# Autodesk Inventor assembly: WCP_DS_-_2_CIM_WCD_Base_Kit_217-3433
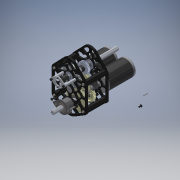
[picture p0: Inventor's stored thumbnail of the model, 180x180]
Saved by Autodesk Inventor 2017 (Build 210142000, 142)
## iProperties
Created: 2013-12-10
Part Number: WCP_DS_-_2_CIM_WCD_Base_Kit_217-3433
Description: STEP AP214
Document SubType Name: Assembly
Designer: 600086
Mass: 1467.69 g
Surface Area: 3535.67 cm^2
Volume: 1467.69 cm^3
Density: 1 g/cm^3
Sending System: SolidWorks 2013
Preprocessor: SwSTEP 2.0
Title: 217-3433-STEP.STEP
Revision Number: ANY
## Documents named in this file (43)
- E:\GrabCAD\Power Hawks CAD\Resources\VEXpro Resources\Gearboxes\WCP shifting Gearbox\WCP_DS_-_2_CIM_WCD_Base_Kit_217-3433.iam
- E:\GrabCAD\Power Hawks CAD\Resources\VEXpro Resources\Gearboxes\WCP shifting Gearbox\217-3423-005 Rev1.ipt
- E:\GrabCAD\Power Hawks CAD\Resources\VEXpro Resources\Gearboxes\WCP shifting Gearbox\217-3195-200 Rev1.iam
- E:\GrabCAD\Power Hawks CAD\Resources\VEXpro Resources\Gearboxes\WCP shifting Gearbox\217-3423-006 Rev1.ipt
- E:\GrabCAD\Power Hawks CAD\Resources\VEXpro Resources\Gearboxes\WCP shifting Gearbox\217-3423-008 Rev1.ipt
- E:\GrabCAD\Power Hawks CAD\Resources\VEXpro Resources\Gearboxes\WCP shifting Gearbox\217-3423-009 Rev1.ipt
- E:\GrabCAD\Power Hawks CAD\Resources\VEXpro Resources\Gearboxes\WCP shifting Gearbox\217-2778-001 Rev2_NCQ8A075-050M.iam
- E:\GrabCAD\Power Hawks CAD\Resources\VEXpro Resources\Gearboxes\WCP shifting Gearbox\217-2731.ipt
- E:\GrabCAD\Power Hawks CAD\Resources\VEXpro Resources\Gearboxes\WCP shifting Gearbox\217-2733.ipt
- E:\GrabCAD\Power Hawks CAD\Resources\VEXpro Resources\Gearboxes\WCP shifting Gearbox\217-2734.ipt
- E:\GrabCAD\Power Hawks CAD\Resources\VEXpro Resources\Gearboxes\WCP shifting Gearbox\217-2743.ipt
- E:\GrabCAD\Power Hawks CAD\Resources\VEXpro Resources\Gearboxes\WCP shifting Gearbox\217-2614-002_98430A132.ipt
- E:\GrabCAD\Power Hawks CAD\Resources\VEXpro Resources\Gearboxes\WCP shifting Gearbox\217-3421-007 Rev1.ipt
- E:\GrabCAD\Power Hawks CAD\Resources\VEXpro Resources\Gearboxes\WCP shifting Gearbox\217-3421-009 Rev1.ipt
- E:\GrabCAD\Power Hawks CAD\Resources\VEXpro Resources\Gearboxes\WCP shifting Gearbox\217-3421-010 Rev1.ipt
- E:\GrabCAD\Power Hawks CAD\Resources\VEXpro Resources\Gearboxes\WCP shifting Gearbox\217-3421-011 Rev2_97633A200.ipt
- E:\GrabCAD\Power Hawks CAD\Resources\VEXpro Resources\Gearboxes\WCP shifting Gearbox\217-3422-007 Rev1.ipt
- E:\GrabCAD\Power Hawks CAD\Resources\VEXpro Resources\Gearboxes\WCP shifting Gearbox\217-3423-014 Rev1.ipt
- E:\GrabCAD\Power Hawks CAD\Resources\VEXpro Resources\Gearboxes\WCP shifting Gearbox\217-3423-016 Rev1.ipt
- E:\GrabCAD\Power Hawks CAD\Resources\VEXpro Resources\Gearboxes\WCP shifting Gearbox\217-3424-003 Rev1.ipt
- E:\GrabCAD\Power Hawks CAD\Resources\VEXpro Resources\Gearboxes\WCP shifting Gearbox\217-2761-001 rev1.ipt
- E:\GrabCAD\Power Hawks CAD\Resources\VEXpro Resources\Gearboxes\WCP shifting Gearbox\217-3210-001 Rev1_30t.ipt
- E:\GrabCAD\Power Hawks CAD\Resources\VEXpro Resources\Gearboxes\WCP shifting Gearbox\217-3215-001 Rev1_42t.ipt
- E:\GrabCAD\Power Hawks CAD\Resources\VEXpro Resources\Gearboxes\WCP shifting Gearbox\217-3414-001 Rev1_14t Steel Pinion.ipt
- E:\GrabCAD\Power Hawks CAD\Resources\VEXpro Resources\Gearboxes\WCP shifting Gearbox\217-3418-001 Rev2_44t.ipt
- E:\GrabCAD\Power Hawks CAD\Resources\VEXpro Resources\Gearboxes\WCP shifting Gearbox\217-3420-001 Rev2_60t.ipt
- E:\GrabCAD\Power Hawks CAD\Resources\VEXpro Resources\Gearboxes\WCP shifting Gearbox\217-3100-001_14t.ipt
- E:\GrabCAD\Power Hawks CAD\Resources\VEXpro Resources\Gearboxes\WCP shifting Gearbox\217-2705-001_30t.ipt
- E:\GrabCAD\Power Hawks CAD\Resources\VEXpro Resources\Gearboxes\WCP shifting Gearbox\217-2000.ipt
- E:\GrabCAD\Power Hawks CAD\Resources\VEXpro Resources\Gearboxes\WCP shifting Gearbox\217-3433-001 Rev1_Default_As Machined_.ipt
- E:\GrabCAD\Power Hawks CAD\Resources\VEXpro Resources\Gearboxes\WCP shifting Gearbox\217-3423-003 Rev1.ipt
- E:\GrabCAD\Power Hawks CAD\Resources\VEXpro Resources\Gearboxes\WCP shifting Gearbox\217-3424-005 Rev1.ipt
- E:\GrabCAD\Power Hawks CAD\Resources\VEXpro Resources\Gearboxes\WCP shifting Gearbox\217-3256-001 Rev1.ipt
- E:\GrabCAD\Power Hawks CAD\Resources\VEXpro Resources\Gearboxes\WCP shifting Gearbox\217-3261-001 Rev1.ipt
- E:\GrabCAD\Power Hawks CAD\Resources\VEXpro Resources\Gearboxes\WCP shifting Gearbox\217-3423-004 Rev1.ipt
- E:\GrabCAD\Power Hawks CAD\Resources\VEXpro Resources\Gearboxes\WCP shifting Gearbox\217-3424-002 Rev1.ipt
- E:\GrabCAD\Power Hawks CAD\Resources\VEXpro Resources\Gearboxes\WCP shifting Gearbox\217-3422-004 Rev2.ipt
- E:\GrabCAD\Power Hawks CAD\Resources\VEXpro Resources\Gearboxes\WCP shifting Gearbox\217-3257-001 Rev1.ipt
- E:\GrabCAD\Power Hawks CAD\Resources\VEXpro Resources\Gearboxes\WCP shifting Gearbox\217-3263-001 Rev1.ipt
- E:\GrabCAD\Power Hawks CAD\Resources\VEXpro Resources\Gearboxes\WCP shifting Gearbox\217-3259-001 Rev1.ipt
- E:\GrabCAD\Power Hawks CAD\Resources\VEXpro Resources\Gearboxes\WCP shifting Gearbox\217-2758-001 Rev1.ipt
- E:\GrabCAD\Power Hawks CAD\Resources\VEXpro Resources\Versa Motion\Sprockets\1.125HexboreSprocket22t-ver-1111-2018.ipt
- E:\GrabCAD\Power Hawks CAD\2018 - Power Up\Chassis\pto\PTO_Add-On_Kit_217-3636.iam
## Components (71 placed, 71 different names)
1. 217-3423-005 Rev1_2 — Rigid:42, Rigid:43, Rigid:44, Rigid:45, Rotational:26
2. 217-3195-200 Rev1_3 [sub-assembly] — Rigid:46
3. 217-3423-006 Rev1_5 — Rigid:45, Rotational:49
4. 217-3423-006 Rev1_6 — Rigid:44, Rotational:48
5. 217-3423-008 Rev1_7 — Mate:4, Mate:5
6. 217-3423-009 Rev1_8 — Rotational:7, Mate:4, Mate:5, Rigid:30, Angle:2, Mate:6
7. 217-2778-001 Rev2_NCQ8A075-050M_9 [sub-assembly] — Rotational:26
8. 217-2731_10 — Rotational:24, Rigid:25, Rigid:29
9. 217-2733_11 — Rotational:4
10. 217-2733_12 — Rotational:2, Rigid:4
11. 217-2734_13 — Rotational:5, Rigid:18, Angle:4
12. 217-2734_14 — Rigid:21, Rigid:22, Cylindrical:1
13. 217-2743_15 — Rigid:24, Rigid:29, Rigid:31
14. 217-2731_16 — Rotational:1
15. 217-2731_17 — Rigid:3
16. 217-2614-002_98430A132_18 — Rigid:34
17. 217-2614-002_98430A132_19 — Rigid:35
18. 217-2614-002_98430A132_20 — Rigid:36
19. 217-2614-002_98430A132_21 — Rigid:37
20. 217-3421-007 Rev1_24 — Rigid:42
21. 217-3421-007 Rev1_25 — Rigid:43
22. 217-3421-009 Rev1_26 — Rigid:51
23. 217-3421-009 Rev1_27 — Rigid:50
24. 217-3421-009 Rev1_28 — Rigid:49
25. 217-3421-009 Rev1_29 — Rigid:52
26. 217-3421-009 Rev1_30 — Rigid:48
27. 217-3421-009 Rev1_31 — Rigid:47
28. 217-3421-010 Rev1_32 — Rigid:40
29. 217-3421-010 Rev1_33 — Rigid:39
30. 217-3421-010 Rev1_34 — Rigid:41
31. 217-3421-010 Rev1_35 — Rigid:38
32. 217-3421-011 Rev2_97633A200_36 — Rigid:26
33. 217-3422-007 Rev1_37 — Mate:7, Flush:3
34. 217-3422-007 Rev1_38 — Mate:8, Flush:2
35. 217-3423-014 Rev1_39 — Rigid:30
36. 217-3423-016 Rev1_40 — Rigid:28
37. 217-3423-016 Rev1_41 — Rigid:27
38. 217-3423-016 Rev1_42
39. 217-3424-003 Rev1_43 — Rigid:14
40. 217-3424-003 Rev1_44 — Rigid:13
41. 217-3424-003 Rev1_45 — Rigid:12
42. 217-3424-003 Rev1_46 — Rigid:11
43. 217-2761-001 rev1_47
44. 217-3210-001 Rev1_30t_50 — Rigid:9
45. 217-3215-001 Rev1_42t_51 — Rigid:8, Rigid:9, Flush:1, Rotation:1, Rotation:2, Rotation:3, Rotation:4
46. 217-3414-001 Rev1_14t Steel Pinion_52217-3414-001 Rev1_14t Steel Pinion_52 — Cylindrical:2, Rigid:34, Rigid:35, Flush:1, Rotation:1
47. 217-3418-001 Rev2_44t_55 — Rigid:24, Rotational:7, Rotation:4
48. 217-3420-001 Rev2_60t_56 — Rigid:21, Mate:6
49. 217-3100-001_14t_57 — Rigid:5, Rigid:7
50. 217-2705-001_30t_58 — Rigid:2, Rigid:53, Rotation:3
51. 217-2000_59 — Rotational:51, Cylindrical:2, Mate:10
52. 217-2000_60 — Rotational:52, Rotational:25, Mate:11
53. 217-3433-001 Rev1_Default<As Machined>_62 — Rotational:4, Rotational:24, Rigid:27, Rigid:28, Rotational:8, Rotational:9, Rotational:52, Rotational:51, Rigid:38, Rigid:39, Rigid:40, Rigid:41, Rotational:48, Rotational:49, Rigid:47, Rigid:48, Mate:10, Mate:11, Rigid:49, Rigid:50, Rigid:51, Rigid:52
54. 217-3433-001 Rev1_Default<As Machined>_63 — Rotational:1, Rotational:2, Mate:1, Mate:2, Mate:3, Rigid:11, Rigid:12, Rigid:13, Rigid:14, Rotational:6, Rigid:15, Rigid:16, Rigid:17, Rotational:56, Rotational:57
55. 217-3423-003 Rev1_64 — Rigid:31, Angle:2, Cylindrical:1, Angle:3, Angle:4, Rigid:46
56. 217-3424-005 Rev1_65 — Rigid:4, Rigid:5
57. 217-3256-001 Rev1_67 — Rigid:7, Rigid:8
58. 217-3261-001 Rev1_68 — Rigid:2, Rigid:3
59. 217-3423-004 Rev1_69 — Rigid:25, Rigid:26
60. 217-3424-002 Rev1_70 — Rigid:17
61. 217-3424-002 Rev1_71 — Rigid:16, Rotational:8
62. 217-3424-002 Rev1_72 — Rotational:6, Rotational:9
63. 217-3424-002 Rev1_73 — Rigid:15
64. 217-3422-004 Rev2_74 — Mate:1, Mate:2, Mate:3, Rotational:5, Mate:7, Mate:8, Flush:2, Flush:3
65. 217-3257-001 Rev1_75 — Rigid:22, Angle:3
66. 217-3263-001 Rev1_76 — Rigid:18, Rigid:19
67. 217-3259-001 Rev1_77 — Rigid:19, Rigid:20
68. 217-2758-001 Rev1_78 — Rigid:20
69. 217-3414-001 Rev1_14t Steel Pinion:2 — Rotational:25, Rigid:36, Rigid:37, Rotation:2
70. 1.125HexboreSprocket22t-ver-1111-2018:1 — Rotational:58, Mate:12
71. PTO_Add-On_Kit_217-3636:1 [sub-assembly] — Rotational:56, Rotational:57, Rigid:53, Rotational:58, Mate:12
## Relationships (88: WeldJoint 47, RevoluteJoint 18, Mate 11, RelateRotation 4, Angle 3, Flush 3, CylindricalJoint 2)
- Rotational:1 [RevoluteJoint]: 217-2731_16 ↔ 217-3433-001 Rev1_Default<As Machined>_63
- Rotational:2 [RevoluteJoint]: 217-2733_12 ↔ 217-3433-001 Rev1_Default<As Machined>_63
- Rigid:2 [WeldJoint]: 217-2705-001_30t_58 ↔ 217-3261-001 Rev1_68
- Rigid:3 [WeldJoint]: 217-2731_17 ↔ 217-3261-001 Rev1_68
- Rigid:4 [WeldJoint]: 217-2733_12 ↔ 217-3424-005 Rev1_65
- Rigid:5 [WeldJoint]: 217-3100-001_14t_57 ↔ 217-3424-005 Rev1_65
- Rotational:4 [RevoluteJoint]: 217-2733_11 ↔ 217-3433-001 Rev1_Default<As Machined>_62
- Rigid:7 [WeldJoint]: 217-3100-001_14t_57 ↔ 217-3256-001 Rev1_67
- Rigid:8 [WeldJoint]: 217-3215-001 Rev1_42t_51 ↔ 217-3256-001 Rev1_67
- Rigid:9 [WeldJoint]: 217-3210-001 Rev1_30t_50 ↔ 217-3215-001 Rev1_42t_51
- Mate:1: 217-3433-001 Rev1_Default<As Machined>_63 ↔ 217-3422-004 Rev2_74
- Mate:2: 217-3433-001 Rev1_Default<As Machined>_63 ↔ 217-3422-004 Rev2_74
- Mate:3: 217-3433-001 Rev1_Default<As Machined>_63 ↔ 217-3422-004 Rev2_74
- Rotational:5 [RevoluteJoint]: 217-2734_13 ↔ 217-3422-004 Rev2_74
- Rigid:11 [WeldJoint]: 217-3424-003 Rev1_46 ↔ 217-3433-001 Rev1_Default<As Machined>_63
- Rigid:12 [WeldJoint]: 217-3424-003 Rev1_45 ↔ 217-3433-001 Rev1_Default<As Machined>_63
- Rigid:13 [WeldJoint]: 217-3424-003 Rev1_44 ↔ 217-3433-001 Rev1_Default<As Machined>_63
- Rigid:14 [WeldJoint]: 217-3424-003 Rev1_43 ↔ 217-3433-001 Rev1_Default<As Machined>_63
- Rotational:6 [RevoluteJoint]: 217-3433-001 Rev1_Default<As Machined>_63 ↔ 217-3424-002 Rev1_72
- Rigid:15 [WeldJoint]: 217-3433-001 Rev1_Default<As Machined>_63 ↔ 217-3424-002 Rev1_73
- Rigid:16 [WeldJoint]: 217-3433-001 Rev1_Default<As Machined>_63 ↔ 217-3424-002 Rev1_71
- Rigid:17 [WeldJoint]: 217-3433-001 Rev1_Default<As Machined>_63 ↔ 217-3424-002 Rev1_70
- Rigid:18 [WeldJoint]: 217-2734_13 ↔ 217-3263-001 Rev1_76
- Rigid:19 [WeldJoint]: 217-3263-001 Rev1_76 ↔ 217-3259-001 Rev1_77
- Rigid:20 [WeldJoint]: 217-3259-001 Rev1_77 ↔ 217-2758-001 Rev1_78
- Rigid:21 [WeldJoint]: 217-2734_14 ↔ 217-3420-001 Rev2_60t_56
- Rigid:22 [WeldJoint]: 217-2734_14 ↔ 217-3257-001 Rev1_75
- Rotational:24 [RevoluteJoint]: 217-2731_10 ↔ 217-3433-001 Rev1_Default<As Machined>_62
- Rigid:24 [WeldJoint]: 217-2743_15 ↔ 217-3418-001 Rev2_44t_55
- Rotational:7 [RevoluteJoint]: 217-3423-009 Rev1_8 ↔ 217-3418-001 Rev2_44t_55
- Rigid:25 [WeldJoint]: 217-2731_10 ↔ 217-3423-004 Rev1_69
- Rigid:26 [WeldJoint]: 217-3421-011 Rev2_97633A200_36 ↔ 217-3423-004 Rev1_69
- Rigid:27 [WeldJoint]: 217-3423-016 Rev1_41 ↔ 217-3433-001 Rev1_Default<As Machined>_62
- Rigid:28 [WeldJoint]: 217-3423-016 Rev1_40 ↔ 217-3433-001 Rev1_Default<As Machined>_62
- Rigid:29 [WeldJoint]: 217-2731_10 ↔ 217-2743_15
- Mate:4: 217-3423-008 Rev1_7 ↔ 217-3423-009 Rev1_8
- Mate:5: 217-3423-008 Rev1_7 ↔ 217-3423-009 Rev1_8
- Rigid:30 [WeldJoint]: 217-3423-009 Rev1_8 ↔ 217-3423-014 Rev1_39
- Rigid:31 [WeldJoint]: 217-2743_15 ↔ 217-3423-003 Rev1_64
- Angle:2 (0 deg): 217-3423-009 Rev1_8 ↔ 217-3423-003 Rev1_64
- Cylindrical:1: 217-2734_14 ↔ 217-3423-003 Rev1_64
- Mate:6 (26.67 mm): 217-3423-009 Rev1_8 ↔ 217-3420-001 Rev2_60t_56
- Angle:3 (0 deg): 217-3423-003 Rev1_64 ↔ 217-3257-001 Rev1_75
- Rotational:8 [RevoluteJoint]: 217-3433-001 Rev1_Default<As Machined>_62 ↔ 217-3424-002 Rev1_71
- Rotational:9 [RevoluteJoint]: 217-3433-001 Rev1_Default<As Machined>_62 ↔ 217-3424-002 Rev1_72
- Rotational:52 [RevoluteJoint]: 217-2000_60 ↔ 217-3433-001 Rev1_Default<As Machined>_62
- Rotational:51 [RevoluteJoint]: 217-2000_59 ↔ 217-3433-001 Rev1_Default<As Machined>_62
- Cylindrical:2: 217-3414-001 Rev1_14t Steel Pinion_52217-3414-001 Rev1_14t Steel Pinion_52 ↔ 217-2000_59
- Rigid:34 [WeldJoint]: 217-2614-002_98430A132_18 ↔ 217-3414-001 Rev1_14t Steel Pinion_52217-3414-001 Rev1_14t Steel Pinion_52
- Rigid:35 [WeldJoint]: 217-2614-002_98430A132_19 ↔ 217-3414-001 Rev1_14t Steel Pinion_52217-3414-001 Rev1_14t Steel Pinion_52
- Flush:1: 217-3215-001 Rev1_42t_51 ↔ 217-3414-001 Rev1_14t Steel Pinion_52217-3414-001 Rev1_14t Steel Pinion_52
- Rotational:25 [RevoluteJoint]: 217-2000_60 ↔ 217-3414-001 Rev1_14t Steel Pinion:2
- Rigid:36 [WeldJoint]: 217-2614-002_98430A132_20 ↔ 217-3414-001 Rev1_14t Steel Pinion:2
- Rigid:37 [WeldJoint]: 217-2614-002_98430A132_21 ↔ 217-3414-001 Rev1_14t Steel Pinion:2
- Mate:7: 217-3422-007 Rev1_37 ↔ 217-3422-004 Rev2_74
- Mate:8: 217-3422-007 Rev1_38 ↔ 217-3422-004 Rev2_74
- Flush:2: 217-3422-007 Rev1_38 ↔ 217-3422-004 Rev2_74
- Flush:3: 217-3422-007 Rev1_37 ↔ 217-3422-004 Rev2_74
- Angle:4 (0 deg): 217-2734_13 ↔ 217-3423-003 Rev1_64
- Rigid:38 [WeldJoint]: 217-3421-010 Rev1_35 ↔ 217-3433-001 Rev1_Default<As Machined>_62
- Rigid:39 [WeldJoint]: 217-3421-010 Rev1_33 ↔ 217-3433-001 Rev1_Default<As Machined>_62
- Rigid:40 [WeldJoint]: 217-3421-010 Rev1_32 ↔ 217-3433-001 Rev1_Default<As Machined>_62
- Rigid:41 [WeldJoint]: 217-3421-010 Rev1_34 ↔ 217-3433-001 Rev1_Default<As Machined>_62
- Rigid:42 [WeldJoint]: 217-3423-005 Rev1_2 ↔ 217-3421-007 Rev1_24
- Rigid:43 [WeldJoint]: 217-3423-005 Rev1_2 ↔ 217-3421-007 Rev1_25
- Rigid:44 [WeldJoint]: 217-3423-005 Rev1_2 ↔ 217-3423-006 Rev1_6
- Rigid:45 [WeldJoint]: 217-3423-005 Rev1_2 ↔ 217-3423-006 Rev1_5
- Rotational:26 [RevoluteJoint]: 217-3423-005 Rev1_2 ↔ 217-2778-001 Rev2_NCQ8A075-050M_9
- Rigid:46 [WeldJoint]: 217-3195-200 Rev1_3 ↔ 217-3423-003 Rev1_64
- Rotational:48 [RevoluteJoint]: 217-3423-006 Rev1_6 ↔ 217-3433-001 Rev1_Default<As Machined>_62
- Rotational:49 [RevoluteJoint]: 217-3423-006 Rev1_5 ↔ 217-3433-001 Rev1_Default<As Machined>_62
- Rigid:47 [WeldJoint]: 217-3421-009 Rev1_31 ↔ 217-3433-001 Rev1_Default<As Machined>_62
- Rigid:48 [WeldJoint]: 217-3421-009 Rev1_30 ↔ 217-3433-001 Rev1_Default<As Machined>_62
- Mate:10: 217-2000_59 ↔ 217-3433-001 Rev1_Default<As Machined>_62
- Mate:11: 217-2000_60 ↔ 217-3433-001 Rev1_Default<As Machined>_62
- Rigid:49 [WeldJoint]: 217-3421-009 Rev1_28 ↔ 217-3433-001 Rev1_Default<As Machined>_62
- Rigid:50 [WeldJoint]: 217-3421-009 Rev1_27 ↔ 217-3433-001 Rev1_Default<As Machined>_62
- Rigid:51 [WeldJoint]: 217-3421-009 Rev1_26 ↔ 217-3433-001 Rev1_Default<As Machined>_62
- Rigid:52 [WeldJoint]: 217-3421-009 Rev1_29 ↔ 217-3433-001 Rev1_Default<As Machined>_62
- Rotational:56 [RevoluteJoint]: 217-3433-001 Rev1_Default<As Machined>_63 ↔ PTO_Add-On_Kit_217-3636:1
- Rotational:57 [RevoluteJoint]: 217-3433-001 Rev1_Default<As Machined>_63 ↔ PTO_Add-On_Kit_217-3636:1
- Rigid:53 [WeldJoint]: 217-2705-001_30t_58 ↔ PTO_Add-On_Kit_217-3636:1
- Rotational:58 [RevoluteJoint]: 1.125HexboreSprocket22t-ver-1111-2018:1 ↔ PTO_Add-On_Kit_217-3636:1
- Mate:12: 1.125HexboreSprocket22t-ver-1111-2018:1 ↔ PTO_Add-On_Kit_217-3636:1
- Rotation:1 [RelateRotation] (1 ul): 217-3215-001 Rev1_42t_51 ↔ 217-3414-001 Rev1_14t Steel Pinion_52217-3414-001 Rev1_14t Steel Pinion_52
- Rotation:2 [RelateRotation] (1 ul): 217-3215-001 Rev1_42t_51 ↔ 217-3414-001 Rev1_14t Steel Pinion:2
- Rotation:3 [RelateRotation] (1 ul): 217-3215-001 Rev1_42t_51 ↔ 217-2705-001_30t_58
- Rotation:4 [RelateRotation] (1 ul): 217-3215-001 Rev1_42t_51 ↔ 217-3418-001 Rev2_44t_55
